# Autodesk Inventor assembly: A Idler
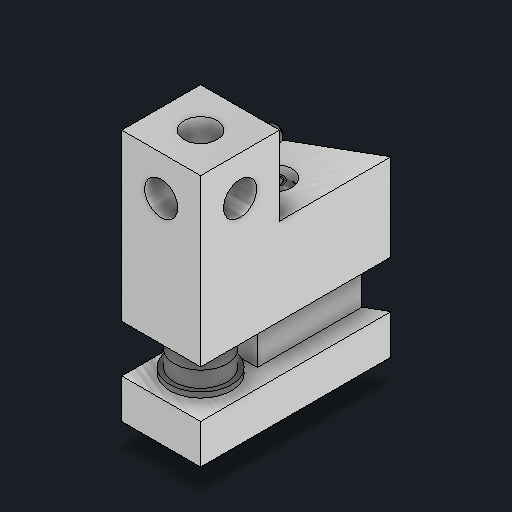
[picture p0: Inventor's stored thumbnail of the model, 512x512]
Saved by Autodesk Inventor 2025.1 (Build 291241020, 241B)
## iProperties
Created: 2025-05-09
Part Number: A Idler
Document SubType Name: Assembly
Designer: AdminForWorker
Title: A Idler
Author: AdminForWorker
## Documents named in this file (6)
- C:\Users\Joshua Eah\Documents\Voron 0.2\CAD\Master Assembly\Motion\Idlers\A Idler.iam
- C:\Users\Joshua Eah\Documents\Voron 0.2\CAD\Machined Parts\Idlers\A Idler\A Idler.ipt
- C:\Users\Joshua Eah\Documents\Voron 0.2\CAD\Master Assembly\Hardware\F623 Stack.iam
- C:\Users\Joshua Eah\Documents\Voron 0.2\CAD\Master Assembly\Hardware\M3 Hexnut.ipt
- C:\Users\Joshua Eah\Documents\Voron 0.2\CAD\Master Assembly\Hardware\M3x10 BHCS.ipt
- C:\Users\Joshua Eah\Documents\Voron 0.2\CAD\Master Assembly\Hardware\M3x35 BHCS.ipt
## Components (6 placed, 5 different names)
1. A Idler:1
2. F623 Stack:1 [sub-assembly]
3. M3 Hexnut:1
4. M3x10 BHCS:1
5. M3x35 BHCS:1
6. M3x35 BHCS:2
## Relationships (1: Insert 1)
- [Insert]: A Idler:1 ↔ M3x10 BHCS:1
